# Autodesk Inventor assembly: reactor sub assem
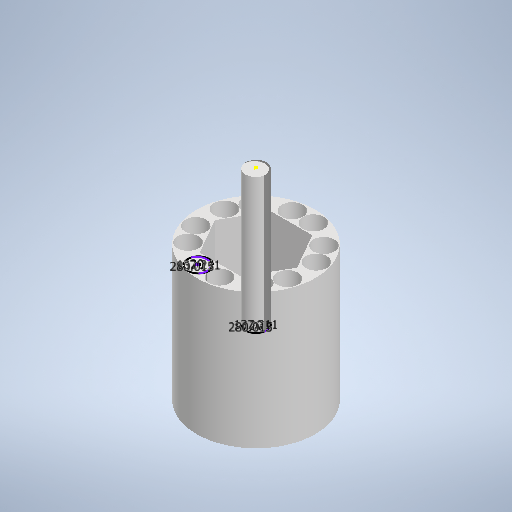
[picture p0: Inventor's stored thumbnail of the model, 512x512]
Saved by Autodesk Inventor 2025.2 (Build 292293000, 293)
## iProperties
Created: 2025-04-28
Part Number: reactor sub assem
Document SubType Name: Assembly
Designer: 5013908
Author: 5013908
## Documents named in this file (3)
- C:\Users\5013908\Documents\GitHub\RAHS-microreactor\reactor sub assem.iam
- C:\Users\5013908\Documents\GitHub\RAHS-microreactor\alumina caseing.ipt
- C:\Users\5013908\Documents\GitHub\RAHS-microreactor\control drum.ipt
## Components (3 placed, 2 different names)
1. alumina caseing:1 — Rotational:1
2. control drum:1
3. control drum:2 — Rotational:1
## Relationships (1: RevoluteJoint 1)
- Rotational:1 [RevoluteJoint]: alumina caseing:1 ↔ control drum:2
